# Autodesk Inventor assembly: fengmingroboticassembly
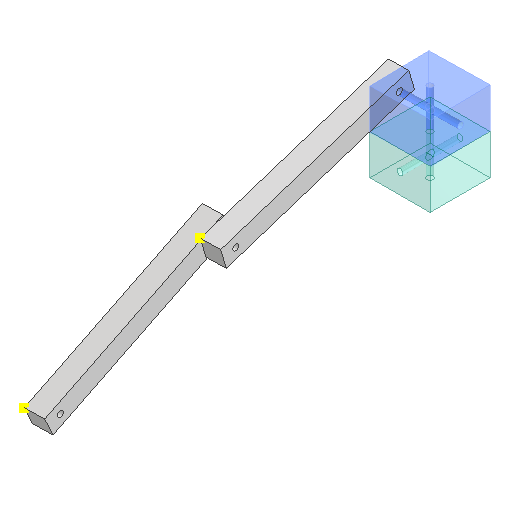
[picture p0: Inventor's stored thumbnail of the model, 512x512]
Saved by Autodesk Inventor 2025 (Build 290162000, 162)
## iProperties
Created: 2025-02-16
Part Number: fengmingroboticassembly
Document SubType Name: Assembly
Designer: wj
Author: wj
## Documents named in this file (3)
- C:\Users\wj\Desktop\fengmingroboticassembly.iam
- C:\Users\wj\Desktop\fengmingroboticarm1.ipt
- C:\Users\wj\Desktop\fengmingroboticarm2.ipt
## Components (4 placed, 2 different names)
1. fengmingroboticarm1:1 — Mate:1, Insert:1, Mate:4, Mate:5
2. fengmingroboticarm1:2 — Mate:1, Insert:1
3. fengmingroboticarm2:1 — Mate:2, Mate:3, Mate:4, Mate:5
4. fengmingroboticarm2:2 — Mate:2, Mate:3
## Relationships (6: Mate 5, Insert 1)
- Mate:1: fengmingroboticarm1:1 ↔ fengmingroboticarm1:2
- Insert:1: fengmingroboticarm1:1 ↔ fengmingroboticarm1:2
- Mate:2: fengmingroboticarm2:1 ↔ fengmingroboticarm2:2
- Mate:3: fengmingroboticarm2:1 ↔ fengmingroboticarm2:2
- Mate:4: fengmingroboticarm1:1 ↔ fengmingroboticarm2:1
- Mate:5: fengmingroboticarm1:1 ↔ fengmingroboticarm2:1
